# Autodesk Inventor assembly: CORL_007_PlanetaryGearbox
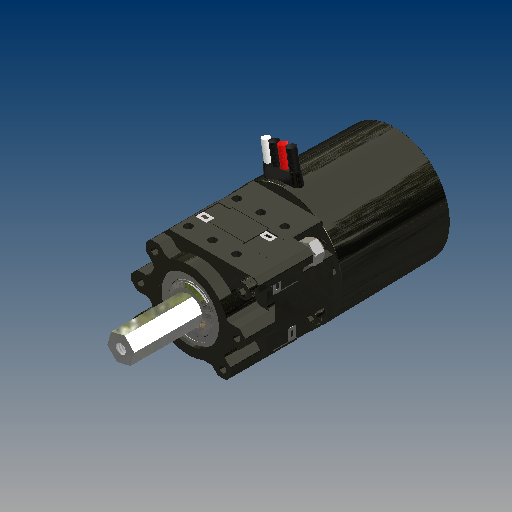
[picture p0: Inventor's stored thumbnail of the model, 512x512]
Saved by Autodesk Inventor 2024.3 (Build 283343000, 343)
## iProperties
Created: 2024-08-02
Part Number: CORL_007_PlanetaryGearbox
Document SubType Name: Assembly
Designer: Bryan
Mass: 880.197 g
Surface Area: 1196.61 cm^2
Volume: 210.345 cm^3
Density: 4.18453 g/cm^3
Author: Bryan
## Documents named in this file (11)
- C:\Users\Kenji\Documents\GitHub\1622-2024-Summer-CAD-A-Thon\Coral\CORL_007_PlanetaryGearbox.iam
- C:\Users\Kenji\Documents\GitHub\1622-2024-Summer-CAD-A-Thon\COTS Library\MAXPlanetary System\COTS_0.5inhexoutput_REV-21-2104.ipt
- C:\Users\Kenji\Documents\GitHub\1622-2024-Summer-CAD-A-Thon\COTS Library\MAXPlanetary System\COTS_InputStage_REV-21-2106.ipt
- C:\Users\Kenji\Documents\GitHub\1622-2024-Summer-CAD-A-Thon\COTS Library\MAXPlanetary System\COTS_NeoShaftAdapter_REV-21-2108.ipt
- C:\Users\Kenji\Documents\GitHub\1622-2024-Summer-CAD-A-Thon\COTS Library\Motors\COTS_REV-21-1650-V1.1_Neo1.1.ipt
- C:\Users\Kenji\Documents\GitHub\1622-2024-Summer-CAD-A-Thon\Coral\CORL_013_SmallShaft.ipt
- C:\Users\Kenji\Documents\GitHub\1622-2024-Summer-CAD-A-Thon\COTS Library\Fasteners\Bolts\Socket-Head\10-32\COTS_91251A342_1-2in Long_Black-Oxide Alloy Steel Socket Head.ipt
- C:\Users\Kenji\Documents\GitHub\1622-2024-Summer-CAD-A-Thon\COTS Library\Fasteners\Bolts\Socket-Head\10-32\COTS_91251A345_Black-Oxide Alloy Steel Socket Head Screw.ipt
- C:\Users\Kenji\Documents\GitHub\1622-2024-Summer-CAD-A-Thon\COTS Library\Fasteners\Bolts\Socket-Head\10-32\COTS_91251A351_Black-Oxide Alloy Steel Socket Head Screw.ipt
- C:\Users\Kenji\Documents\GitHub\1622-2024-Summer-CAD-A-Thon\COTS Library\Fasteners\Nuts\COTS_90631A411_10-32_Nylock_Nut.ipt
- C:\Users\Kenji\Documents\GitHub\1622-2024-Summer-CAD-A-Thon\COTS Library\MAXPlanetary System\COTS_5to1Stage_REV-21-2103.ipt
## Components (13 placed, 10 different names)
1. COTS_0.5inhexoutput_REV-21-2104:1 — Mate:10, Mate:11, Mate:13, Mate:18, Mate:19, Mate:20, Mate:21, Mate:29, Flush:2
2. COTS_InputStage_REV-21-2106:1 — Mate:5, Mate:8, Mate:9, Mate:14, Mate:15, Mate:16, Mate:17, Mate:23, Mate:25, Mate:27, Flush:1, Mate:28
3. COTS_NeoShaftAdapter_REV-21-2108:1 — Mate:5, Mate:7
4. COTS_REV-21-1650-V1.1_Neo1.1:1 — Mate:7, Mate:8, Mate:9
5. CORL_013_SmallShaft:1 — Mate:10, Mate:11, Mate:12
6. COTS_91251A345_Black-Oxide Alloy Steel Socket Head Screw:1 — Mate:12, Mate:13
7. COTS_91251A342_1-2in Long_Black-Oxide Alloy Steel Socket Head:1 — Mate:14, Mate:17
8. COTS_91251A342_1-2in Long_Black-Oxide Alloy Steel Socket Head:2 — Mate:15, Mate:16
9. COTS_91251A351_Black-Oxide Alloy Steel Socket Head Screw:1 — Mate:18, Mate:21, Mate:22
10. COTS_91251A351_Black-Oxide Alloy Steel Socket Head Screw:2 — Mate:19, Mate:20, Mate:24, Mate:26, Mate:27
11. COTS_90631A411_10-32_Nylock_Nut:1 — Mate:22, Mate:23
12. COTS_90631A411_10-32_Nylock_Nut:2 — Mate:24, Mate:25
13. COTS_5to1Stage_REV-21-2103:1 — Mate:26, Flush:1, Mate:28, Mate:29, Flush:2
## Relationships (26: Mate 24, Flush 2)
- Mate:5: COTS_InputStage_REV-21-2106:1 ↔ COTS_NeoShaftAdapter_REV-21-2108:1
- Mate:7: COTS_NeoShaftAdapter_REV-21-2108:1 ↔ COTS_REV-21-1650-V1.1_Neo1.1:1
- Mate:8: COTS_InputStage_REV-21-2106:1 ↔ COTS_REV-21-1650-V1.1_Neo1.1:1
- Mate:9: COTS_InputStage_REV-21-2106:1 ↔ COTS_REV-21-1650-V1.1_Neo1.1:1
- Mate:10: COTS_0.5inhexoutput_REV-21-2104:1 ↔ CORL_013_SmallShaft:1
- Mate:11: COTS_0.5inhexoutput_REV-21-2104:1 ↔ CORL_013_SmallShaft:1
- Mate:12: CORL_013_SmallShaft:1 ↔ COTS_91251A345_Black-Oxide Alloy Steel Socket Head Screw:1
- Mate:13: COTS_0.5inhexoutput_REV-21-2104:1 ↔ COTS_91251A345_Black-Oxide Alloy Steel Socket Head Screw:1
- Mate:14: COTS_InputStage_REV-21-2106:1 ↔ COTS_91251A342_1-2in Long_Black-Oxide Alloy Steel Socket Head:1
- Mate:15: COTS_InputStage_REV-21-2106:1 ↔ COTS_91251A342_1-2in Long_Black-Oxide Alloy Steel Socket Head:2
- Mate:16: COTS_InputStage_REV-21-2106:1 ↔ COTS_91251A342_1-2in Long_Black-Oxide Alloy Steel Socket Head:2
- Mate:17: COTS_InputStage_REV-21-2106:1 ↔ COTS_91251A342_1-2in Long_Black-Oxide Alloy Steel Socket Head:1
- Mate:18: COTS_0.5inhexoutput_REV-21-2104:1 ↔ COTS_91251A351_Black-Oxide Alloy Steel Socket Head Screw:1
- Mate:19: COTS_0.5inhexoutput_REV-21-2104:1 ↔ COTS_91251A351_Black-Oxide Alloy Steel Socket Head Screw:2
- Mate:20: COTS_0.5inhexoutput_REV-21-2104:1 ↔ COTS_91251A351_Black-Oxide Alloy Steel Socket Head Screw:2
- Mate:21: COTS_0.5inhexoutput_REV-21-2104:1 ↔ COTS_91251A351_Black-Oxide Alloy Steel Socket Head Screw:1
- Mate:22: COTS_91251A351_Black-Oxide Alloy Steel Socket Head Screw:1 ↔ COTS_90631A411_10-32_Nylock_Nut:1
- Mate:23: COTS_InputStage_REV-21-2106:1 ↔ COTS_90631A411_10-32_Nylock_Nut:1
- Mate:24: COTS_91251A351_Black-Oxide Alloy Steel Socket Head Screw:2 ↔ COTS_90631A411_10-32_Nylock_Nut:2
- Mate:25: COTS_InputStage_REV-21-2106:1 ↔ COTS_90631A411_10-32_Nylock_Nut:2
- Mate:26: COTS_91251A351_Black-Oxide Alloy Steel Socket Head Screw:2 ↔ COTS_5to1Stage_REV-21-2103:1
- Mate:27: COTS_InputStage_REV-21-2106:1 ↔ COTS_91251A351_Black-Oxide Alloy Steel Socket Head Screw:2
- Flush:1: COTS_InputStage_REV-21-2106:1 ↔ COTS_5to1Stage_REV-21-2103:1
- Mate:28: COTS_InputStage_REV-21-2106:1 ↔ COTS_5to1Stage_REV-21-2103:1
- Mate:29: COTS_0.5inhexoutput_REV-21-2104:1 ↔ COTS_5to1Stage_REV-21-2103:1
- Flush:2: COTS_0.5inhexoutput_REV-21-2104:1 ↔ COTS_5to1Stage_REV-21-2103:1
